# Autodesk Inventor assembly: USB Cable B Male to B Female 90 degrees_Assembly
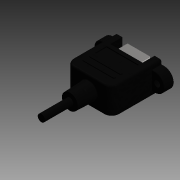
[picture p0: Inventor's stored thumbnail of the model, 180x180]
Saved by Autodesk Inventor 2016 (Build 200138000, 138)
## iProperties
Created: 2017-10-16
Part Number: USB Cable B Male to B Female 90 degrees_Assembly
Document SubType Name: Assembly
Designer: admin
Author: admin
## Documents named in this file (3)
- D:\Dropbox\CAD\Kossel2\CAD\USB Cable B Male to B Female 90 degrees_Assembly.iam
- D:\Dropbox\CAD\Kossel2\CAD\USB Cable B Male to B Female 90 degrees.ipt
- D:\Dropbox\CAD\Kossel2\CAD\USB B Female Port.ipt
## Components (2 placed, 2 different names)
1. USB Cable B Male to B Female 90 degrees:1 — Flush:1, Flush:2, Mate:1
2. USB B Female Port:1 — Flush:1, Flush:2, Mate:1
## Relationships (3: Flush 2, Mate 1)
- Flush:1 (1.6135 mm): USB Cable B Male to B Female 90 degrees:1 ↔ USB B Female Port:1
- Flush:2 (-6.41 mm): USB Cable B Male to B Female 90 degrees:1 ↔ USB B Female Port:1
- Mate:1 (2.4675 mm): USB Cable B Male to B Female 90 degrees:1 ↔ USB B Female Port:1
